# Autodesk Inventor assembly: Assembly
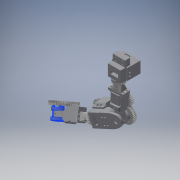
[picture p0: Inventor's stored thumbnail of the model, 180x180]
Saved by Autodesk Inventor 2019 (Build 230136000, 136)
## iProperties
Created: 2020-04-08
Part Number: Assembly
Document SubType Name: Assembly
Designer: isaac
Author: isaac
## Documents named in this file (10)
- C:\2_Development\Robot_arm\Assembly.iam
- C:\2_Development\Robot_arm\Swivel Joint Driver.ipt
- C:\2_Development\Robot_arm\Swivel Joint Driven.ipt
- C:\2_Development\Robot_arm\Servo Joint.ipt
- C:\2_Development\Robot_arm\Arm Joint.ipt
- C:\2_Development\Robot_arm\LX-16A.ipt
- C:\2_Development\Robot_arm\Swivel Joint Servo Gear.ipt
- C:\2_Development\Robot_arm\Double Helix Driven Gear.ipt
- C:\2_Development\Robot_arm\Double Helix Servo Gear.ipt
- C:\2_Development\Robot_arm\Swivel Arm Servo Holder.ipt
## Components (20 placed, 7 different names)
1. Swivel Joint Driver:1 — Mate:1, Mate:2, Mate:18, Flush:1, Flush:2, Mate:41, Mate:42, Mate:43
2. Spur Gear2:1 — Mate:1, Mate:2, Mate:3, Mate:4, Mate:5, Rotation:1
3. Servo Joint:1 — Mate:3, Mate:4, Mate:5, Mate:6, Mate:7, Mate:21, Mate:22, Mate:23
4. Arm Joint:1 — Mate:6, Mate:7, Mate:8, Mate:9, Mate:10, Mate:24, Mate:25, Rotation:2
5. Swivel Joint Driver:2 — Mate:8, Mate:9, Mate:10, Mate:11, Mate:12, Mate:26, Flush:3, Flush:4, Mate:38, Mate:39, Mate:40
6. Spur Gear2:2 — Mate:11, Mate:12, Mate:13, Mate:14, Mate:15, Rotation:5
7. Servo Joint:2 — Mate:13, Mate:14, Mate:15, Mate:16, Mate:17, Mate:27, Mate:28, Mate:29
8. Arm Joint:2 — Mate:16, Mate:17, Mate:30, Mate:31, Rotation:3
9. LX-16A:1 — Mate:18, Flush:1, Mate:19, Mate:20, Flush:2
10. LX-16A:2 — Mate:21, Mate:22, Mate:23, Mate:32, Mate:33
11. LX-16A:3 — Mate:26, Flush:3, Flush:4, Mate:34, Mate:35
12. LX-16A:4 — Mate:27, Mate:28, Mate:29, Mate:36, Mate:37
13. Spur Gear1:1 — Mate:19, Mate:20, Rotation:1
14. Spur Gear2:3 — Mate:24, Mate:25, Rotation:2, Rotation:4
15. Spur Gear2:4 — Mate:30, Mate:31, Rotation:3, Rotation:6
16. Spur Gear1:2 — Mate:32, Mate:33, Rotation:4
17. Spur Gear1:3 — Mate:34, Mate:35, Rotation:5
18. Spur Gear1:4 — Mate:36, Mate:37, Rotation:6
19. Swivel Arm Servo Holder:1 — Mate:38, Mate:39, Mate:40
20. Swivel Arm Servo Holder:2 — Mate:41, Mate:42, Mate:43
## Relationships (53: Mate 43, RelateRotation 6, Flush 4)
- Mate:1: Swivel Joint Driver:1 ↔ Spur Gear2:1
- Mate:2 (0.4 mm): Swivel Joint Driver:1 ↔ Spur Gear2:1
- Mate:3: Spur Gear2:1 ↔ Servo Joint:1
- Mate:4: Spur Gear2:1 ↔ Servo Joint:1
- Mate:5: Spur Gear2:1 ↔ Servo Joint:1
- Mate:6 (0.25 mm): Servo Joint:1 ↔ Arm Joint:1
- Mate:7: Servo Joint:1 ↔ Arm Joint:1
- Mate:8: Arm Joint:1 ↔ Swivel Joint Driver:2
- Mate:9: Arm Joint:1 ↔ Swivel Joint Driver:2
- Mate:10: Arm Joint:1 ↔ Swivel Joint Driver:2
- Mate:11 (0.4 mm): Swivel Joint Driver:2 ↔ Spur Gear2:2
- Mate:12: Swivel Joint Driver:2 ↔ Spur Gear2:2
- Mate:13: Spur Gear2:2 ↔ Servo Joint:2
- Mate:14: Spur Gear2:2 ↔ Servo Joint:2
- Mate:15: Spur Gear2:2 ↔ Servo Joint:2
- Mate:16 (0.25 mm): Servo Joint:2 ↔ Arm Joint:2
- Mate:17: Servo Joint:2 ↔ Arm Joint:2
- Mate:18: Swivel Joint Driver:1 ↔ LX-16A:1
- Flush:1: Swivel Joint Driver:1 ↔ LX-16A:1
- Mate:19: LX-16A:1 ↔ Spur Gear1:1
- Mate:20: LX-16A:1 ↔ Spur Gear1:1
- Flush:2: Swivel Joint Driver:1 ↔ LX-16A:1
- Rotation:1 [RelateRotation] (1 ul): Spur Gear2:1 ↔ Spur Gear1:1
- Mate:21: Servo Joint:1 ↔ LX-16A:2
- Mate:22: Servo Joint:1 ↔ LX-16A:2
- Mate:23: Servo Joint:1 ↔ LX-16A:2
- Mate:24: Arm Joint:1 ↔ Spur Gear2:3
- Mate:25: Arm Joint:1 ↔ Spur Gear2:3
- Rotation:2 [RelateRotation] (1 ul): Arm Joint:1 ↔ Spur Gear2:3
- Mate:26: Swivel Joint Driver:2 ↔ LX-16A:3
- Flush:3: Swivel Joint Driver:2 ↔ LX-16A:3
- Flush:4: Swivel Joint Driver:2 ↔ LX-16A:3
- Mate:27: Servo Joint:2 ↔ LX-16A:4
- Mate:28: Servo Joint:2 ↔ LX-16A:4
- Mate:29: Servo Joint:2 ↔ LX-16A:4
- Mate:30: Arm Joint:2 ↔ Spur Gear2:4
- Mate:31: Arm Joint:2 ↔ Spur Gear2:4
- Rotation:3 [RelateRotation] (1 ul): Arm Joint:2 ↔ Spur Gear2:4
- Mate:32: LX-16A:2 ↔ Spur Gear1:2
- Mate:33: LX-16A:2 ↔ Spur Gear1:2
- Rotation:4 [RelateRotation] (0.666 ul): Spur Gear2:3 ↔ Spur Gear1:2
- Mate:34: LX-16A:3 ↔ Spur Gear1:3
- Mate:35: LX-16A:3 ↔ Spur Gear1:3
- Rotation:5 [RelateRotation] (1 ul): Spur Gear2:2 ↔ Spur Gear1:3
- Mate:36: LX-16A:4 ↔ Spur Gear1:4
- Mate:37: LX-16A:4 ↔ Spur Gear1:4
- Rotation:6 [RelateRotation] (1.5 ul): Spur Gear2:4 ↔ Spur Gear1:4
- Mate:38: Swivel Joint Driver:2 ↔ Swivel Arm Servo Holder:1
- Mate:39: Swivel Joint Driver:2 ↔ Swivel Arm Servo Holder:1
- Mate:40: Swivel Joint Driver:2 ↔ Swivel Arm Servo Holder:1
- Mate:41: Swivel Joint Driver:1 ↔ Swivel Arm Servo Holder:2
- Mate:42: Swivel Joint Driver:1 ↔ Swivel Arm Servo Holder:2
- Mate:43: Swivel Joint Driver:1 ↔ Swivel Arm Servo Holder:2
